# Autodesk Inventor assembly: az_rot_plate
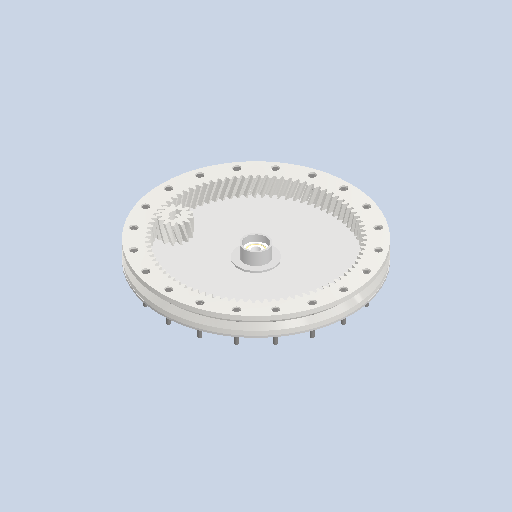
[picture p0: Inventor's stored thumbnail of the model, 512x512]
Saved by Autodesk Inventor 2024 (Build 280153000, 153)
## iProperties
Created: 2025-12-10
Part Number: az_rot_plate
Document SubType Name: Assembly
Designer: schar
Author: schar
## Documents named in this file (7)
- C:\Users\schar\Desktop\projectBlueprint\AMSTS\hardware\az_rot_plate.iam
- C:\Users\schar\Desktop\projectBlueprint\AMSTS\hardware\baseplate_azimuth_gear.ipt
- C:\Users\schar\Desktop\projectBlueprint\AMSTS\hardware\foot_bearings_holder.ipt
- C:\Users\schar\Desktop\projectBlueprint\AMSTS\hardware\azimuth_gear.iam
- C:\Users\schar\Documents\Inventor\Content Center Files\R2024\en-US\AS 1420\AS 1420 - 1973 - M4 x 30.ipt
- C:\Users\schar\Desktop\projectBlueprint\AMSTS\hardware\609_bearing.ipt
- C:\Users\schar\Desktop\projectBlueprint\AMSTS\hardware\6901_bearing.iam
## Components (25 placed, 6 different names)
1. baseplate_azimuth_gear:1 — Mate:1, Mate:2, Mate:11, Mate:12
2. foot_bearings_holder:1 — Mate:1, Mate:2, Mate:7, Mate:8
3. azimuth_gear:1 [sub-assembly] — Mate:5, Mate:6, Mate:11, Mate:12
4. 609_bearing:1 — Mate:7, Mate:8, Mate:9, Mate:10
5. 6901_bearing:1 [sub-assembly] — Mate:9, Mate:10
6. AS 1420 - Metric M4 x 30:1 — Mate:5, Mate:6
7. AS 1420 - Metric M4 x 30:2
8. AS 1420 - Metric M4 x 30:3
9. AS 1420 - Metric M4 x 30:4
10. AS 1420 - Metric M4 x 30:5
11. AS 1420 - Metric M4 x 30:6
12. AS 1420 - Metric M4 x 30:7
13. AS 1420 - Metric M4 x 30:8
14. AS 1420 - Metric M4 x 30:9
15. AS 1420 - Metric M4 x 30:10
16. AS 1420 - Metric M4 x 30:11
17. AS 1420 - Metric M4 x 30:12
18. AS 1420 - Metric M4 x 30:13
19. AS 1420 - Metric M4 x 30:14
20. AS 1420 - Metric M4 x 30:15
21. AS 1420 - Metric M4 x 30:16
22. AS 1420 - Metric M4 x 30:17
23. AS 1420 - Metric M4 x 30:18
24. AS 1420 - Metric M4 x 30:19
25. AS 1420 - Metric M4 x 30:20
## Component patterns: (20 elements, first: AS 1420 - Metric M4 x 30:1)
## Relationships (10: Mate 10)
- Mate:1: baseplate_azimuth_gear:1 ↔ foot_bearings_holder:1
- Mate:2: baseplate_azimuth_gear:1 ↔ foot_bearings_holder:1
- Mate:5: azimuth_gear:1 ↔ AS 1420 - Metric M4 x 30:1
- Mate:6: azimuth_gear:1 ↔ AS 1420 - Metric M4 x 30:1
- Mate:7: foot_bearings_holder:1 ↔ 609_bearing:1
- Mate:8: foot_bearings_holder:1 ↔ 609_bearing:1
- Mate:9: 609_bearing:1 ↔ 6901_bearing:1
- Mate:10: 609_bearing:1 ↔ 6901_bearing:1
- Mate:11: baseplate_azimuth_gear:1 ↔ azimuth_gear:1
- Mate:12: baseplate_azimuth_gear:1 ↔ azimuth_gear:1
